# Autodesk Inventor assembly: Сборка3
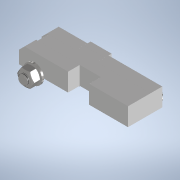
[picture p0: Inventor's stored thumbnail of the model, 180x180]
Saved by Autodesk Inventor 2022 (Build 260153000, 153)
## iProperties
Created: 2024-04-27
Part Number: Сборка3
Document SubType Name: Assembly
Designer: Pavel
Mass: 402.99 g
Surface Area: 627.54 cm^2
Volume: 275.225 cm^3
Density: 1.46422 g/cm^3
Author: Pavel
## Documents named in this file (9)
- D:\BSUIR\KMEKES\Сборка3.iam
- D:\BSUIR\KMEKES\Деталь1.ipt
- C:\Users\Pavel\Documents\Inventor\Content Center Files\R2022\ru-RU\GOST 11371-78  A\Шайба 12 ГОСТ 11371-78.ipt
- C:\Users\Pavel\Documents\Inventor\Content Center Files\R2022\ru-RU\GOST 5915-70\Гайка M12-6H ГОСТ 5915-70(1).ipt
- C:\Users\Pavel\Documents\Inventor\Content Center Files\R2022\ru-RU\Bolt GOST 7798-78\Болт M12-6g×60 ГОСТ 7798-70.ipt
- C:\Users\Pavel\Documents\Inventor\Content Center Files\R2022\ru-RU\Screw A GOST 17473-80\Винт A.M8-6gx25 ГОСТ 17473-80.ipt
- C:\Users\Pavel\Documents\Inventor\Content Center Files\R2022\ru-RU\Stud GOST 22032-76\Шпилька M10-6g×30 ГОСТ 22032-76.ipt
- C:\Users\Pavel\Documents\Inventor\Content Center Files\R2022\ru-RU\Washer 1 GOST 6402-78\Шайба 10Н ГОСТ 6402-78.ipt
- C:\Users\Pavel\Documents\Inventor\Content Center Files\R2022\ru-RU\GOST 5915-70\Гайка M10-6H ГОСТ 5915-70(1).ipt
## Components (8 placed, 8 different names)
1. Деталь1:1 — Вставка:6, Совмещение:9, Совмещение:10, Вставка:8, Вставка:9
2. Болт ГОСТ 7798-70 M12-6g×60:1 — Вставка:6, Касательность:1, Вставка:7, Совмещение:7
3. Шайба  ГОСТ 11371-78 13:1 — Касательность:1, Вставка:7, Совмещение:8
4. Гайка ГОСТ 5915-70 M12:1 — Совмещение:7, Совмещение:8
5. Винт A ГОСТ 17473-80 M8-6gx25:1 — Совмещение:9, Совмещение:10
6. Шпилька ГОСТ 22032-76 M10-6g×30:1 — Вставка:8
7. Шайба 1 ГОСТ 6402-78 10Н:1 — Вставка:9, Вставка:10
8. Гайка ГОСТ 5915-70 M10:1 — Вставка:10
## Relationships (10: Insert 5, Mate 4, Tangent 1)
- Вставка:6 [Insert]: Деталь1:1 ↔ Болт ГОСТ 7798-70 M12-6g×60:1
- Касательность:1 [Tangent]: Болт ГОСТ 7798-70 M12-6g×60:1 ↔ Шайба  ГОСТ 11371-78 13:1
- Вставка:7 [Insert] (-15 mm): Болт ГОСТ 7798-70 M12-6g×60:1 ↔ Шайба  ГОСТ 11371-78 13:1
- Совмещение:7 [Mate]: Болт ГОСТ 7798-70 M12-6g×60:1 ↔ Гайка ГОСТ 5915-70 M12:1
- Совмещение:8 [Mate]: Шайба  ГОСТ 11371-78 13:1 ↔ Гайка ГОСТ 5915-70 M12:1
- Совмещение:9 [Mate]: Деталь1:1 ↔ Винт A ГОСТ 17473-80 M8-6gx25:1
- Совмещение:10 [Mate]: Деталь1:1 ↔ Винт A ГОСТ 17473-80 M8-6gx25:1
- Вставка:8 [Insert] (-10 mm): Деталь1:1 ↔ Шпилька ГОСТ 22032-76 M10-6g×30:1
- Вставка:9 [Insert]: Деталь1:1 ↔ Шайба 1 ГОСТ 6402-78 10Н:1
- Вставка:10 [Insert]: Шайба 1 ГОСТ 6402-78 10Н:1 ↔ Гайка ГОСТ 5915-70 M10:1
